# Autodesk Inventor assembly: リンク_6_1
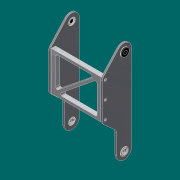
[picture p0: Inventor's stored thumbnail of the model, 180x180]
Saved by Autodesk Inventor 2016 (Build 200138000, 138)
## iProperties
Created: 2016-08-23
Part Number: リンク_6_1
Material: 一般
Document SubType Name: Assembly
Designer: hiro
Mass: 33.5175 g
Surface Area: 182.778 cm^2
Volume: 15.549 cm^3
Density: 2.15561 g/cm^3
Author: hiro
## Documents named in this file (5)
- C:\Users\hiro\Documents\kenkyuu\二足\二足ver6.0\下半身_160823\リンク\リンク_6_2.iam
- C:\Users\hiro\Documents\kenkyuu\二足\二足ver6.0\既製品\NSK_RB_MF85ZZ\MF85ZZ.iam
- C:\Users\hiro\Documents\kenkyuu\二足\二足ver6.0\下半身_160823\リンク\リンク_メインフレーム_6_2.ipt
- C:\Users\hiro\Documents\kenkyuu\二足\二足ver6.0\下半身\リンク\ふくらはぎ\リンク_ふくらはぎ_サブフレーム_1_1(予備案).ipt
- C:\Users\hiro\Documents\kenkyuu\二足\二足ver6.0\既製品\新規購入\D4050-9120B.ipt
## Components (9 placed, 4 different names)
1. MF85ZZ:1 [sub-assembly] — 挿入:13
2. MF85ZZ:2 [sub-assembly] — 挿入:2
3. リンク_メインフレーム_6_2:1 — 挿入:2, 挿入:17, 挿入:18, 挿入:19, 挿入:21
4. リンク_メインフレーム_6_2:2 — 挿入:13, 挿入:14, 挿入:15, 挿入:16, 挿入:20
5. リンク_ふくらはぎ_サブフレーム_1_1(予備案):1 — 挿入:14, 挿入:15, 挿入:16, 挿入:17, 挿入:18, 挿入:19
6. MF85ZZ:3 [sub-assembly] — 挿入:20, 挿入:22
7. MF85ZZ:4 [sub-assembly] — 挿入:21, 挿入:23
8. D4050-9120B:1 — 挿入:22
9. D4050-9120B:2 — 挿入:23
## Relationships (12: Insert 12)
- 挿入:2 [Insert]: MF85ZZ:2 ↔ リンク_メインフレーム_6_2:1
- 挿入:13 [Insert]: MF85ZZ:1 ↔ リンク_メインフレーム_6_2:2
- 挿入:14 [Insert]: リンク_メインフレーム_6_2:2 ↔ リンク_ふくらはぎ_サブフレーム_1_1(予備案):1
- 挿入:15 [Insert]: リンク_メインフレーム_6_2:2 ↔ リンク_ふくらはぎ_サブフレーム_1_1(予備案):1
- 挿入:16 [Insert]: リンク_メインフレーム_6_2:2 ↔ リンク_ふくらはぎ_サブフレーム_1_1(予備案):1
- 挿入:17 [Insert]: リンク_メインフレーム_6_2:1 ↔ リンク_ふくらはぎ_サブフレーム_1_1(予備案):1
- 挿入:18 [Insert]: リンク_メインフレーム_6_2:1 ↔ リンク_ふくらはぎ_サブフレーム_1_1(予備案):1
- 挿入:19 [Insert]: リンク_メインフレーム_6_2:1 ↔ リンク_ふくらはぎ_サブフレーム_1_1(予備案):1
- 挿入:20 [Insert]: リンク_メインフレーム_6_2:2 ↔ MF85ZZ:3
- 挿入:21 [Insert]: リンク_メインフレーム_6_2:1 ↔ MF85ZZ:4
- 挿入:22 [Insert]: MF85ZZ:3 ↔ D4050-9120B:1
- 挿入:23 [Insert]: MF85ZZ:4 ↔ D4050-9120B:2
